# Autodesk Inventor assembly: StorageAssembly.ver4-1111-2020
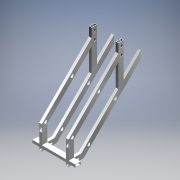
[picture p0: Inventor's stored thumbnail of the model, 180x180]
Saved by Autodesk Inventor 2018 (Build 220112000, 112)
## iProperties
Created: 2020-01-21
Part Number: StorageAssembly.ver4-1111-2020
Document SubType Name: Assembly
Designer: Power Hawks CADD
Author: Power Hawks CADD
## Documents named in this file (7)
- E:\GrabCAD\Power Hawks CAD\2020 Infinite Recharge\Storage\Assemblies\StorageAssembly.ver4-1111-2020.iam
- E:\GrabCAD\Power Hawks CAD\2020 Infinite Recharge\Shooting\Parts\SmallAnglesSupport.ver1-1111-2020.ipt
- E:\GrabCAD\Power Hawks CAD\2020 Infinite Recharge\Shooting\Parts\SmallAnglesSupport.ver1-1111-2020_MIR.ipt
- E:\GrabCAD\Power Hawks CAD\2020 Infinite Recharge\Storage\Assemblies\StorageAssembly.ver3-1111-2020.iam
- E:\GrabCAD\Power Hawks CAD\2020 Infinite Recharge\Storage\Parts\IntakeBrace.ver1-1111-2020.ipt
- E:\GrabCAD\Power Hawks CAD\2020 Infinite Recharge\Storage\Parts\StorageSupport.ver1-1111-2020.ipt
- E:\GrabCAD\Power Hawks CAD\2020 Infinite Recharge\Storage\Parts\AngleBrace.ver2-1111-2020.ipt
## Components (8 placed, 6 different names)
1. SmallAnglesSupport.ver1-1111-2020:1 — Mate:10, Mate:16, Mate:18, Flush:18, Flush:19, Flush:23, Flush:29
2. SmallAnglesSupport.ver1-1111-2020_MIR:1 — Mate:12, Flush:13, Flush:14, Mate:16, Mate:21, Flush:21, Flush:22, Flush:24
3. StorageAssembly.ver3-1111-2020:1 [sub-assembly] — Flush:12, Flush:13, Mate:17, Mate:23, Mate:25, Mate:26
4. IntakeBrace.ver1-1111-2020:1 — Mate:10, Flush:12, Mate:12, Flush:14, Mate:17, Angle:1, Flush:23, Flush:24, Flush:29
5. StorageSupport.ver1-1111-2020:1 — Flush:28, Mate:26, Mate:28
6. StorageSupport.ver1-1111-2020:2 — Flush:27, Mate:25, Mate:27
7. AngleBrace.ver2-1111-2020:1 — Mate:18, Flush:18, Flush:19, Flush:27, Mate:27
8. AngleBrace.ver2-1111-2020:2 — Mate:21, Flush:21, Flush:22, Flush:28, Mate:28
## Relationships (24: Flush 12, Mate 11, Angle 1)
- Mate:10: SmallAnglesSupport.ver1-1111-2020:1 ↔ IntakeBrace.ver1-1111-2020:1
- Flush:12: StorageAssembly.ver3-1111-2020:1 ↔ IntakeBrace.ver1-1111-2020:1
- Mate:12: SmallAnglesSupport.ver1-1111-2020_MIR:1 ↔ IntakeBrace.ver1-1111-2020:1
- Flush:13: SmallAnglesSupport.ver1-1111-2020_MIR:1 ↔ StorageAssembly.ver3-1111-2020:1
- Flush:14: SmallAnglesSupport.ver1-1111-2020_MIR:1 ↔ IntakeBrace.ver1-1111-2020:1
- Mate:16 (228.6 mm): SmallAnglesSupport.ver1-1111-2020:1 ↔ SmallAnglesSupport.ver1-1111-2020_MIR:1
- Mate:17: StorageAssembly.ver3-1111-2020:1 ↔ IntakeBrace.ver1-1111-2020:1
- Mate:18: SmallAnglesSupport.ver1-1111-2020:1 ↔ AngleBrace.ver2-1111-2020:1
- Flush:18: SmallAnglesSupport.ver1-1111-2020:1 ↔ AngleBrace.ver2-1111-2020:1
- Flush:19: SmallAnglesSupport.ver1-1111-2020:1 ↔ AngleBrace.ver2-1111-2020:1
- Mate:21: SmallAnglesSupport.ver1-1111-2020_MIR:1 ↔ AngleBrace.ver2-1111-2020:2
- Flush:21: SmallAnglesSupport.ver1-1111-2020_MIR:1 ↔ AngleBrace.ver2-1111-2020:2
- Flush:22: SmallAnglesSupport.ver1-1111-2020_MIR:1 ↔ AngleBrace.ver2-1111-2020:2
- Angle:1 (0 deg): IntakeBrace.ver1-1111-2020:1
- Flush:23: SmallAnglesSupport.ver1-1111-2020:1 ↔ IntakeBrace.ver1-1111-2020:1
- Flush:24: SmallAnglesSupport.ver1-1111-2020_MIR:1 ↔ IntakeBrace.ver1-1111-2020:1
- Mate:23: StorageAssembly.ver3-1111-2020:1
- Flush:27: StorageSupport.ver1-1111-2020:2 ↔ AngleBrace.ver2-1111-2020:1
- Mate:25: StorageAssembly.ver3-1111-2020:1 ↔ StorageSupport.ver1-1111-2020:2
- Flush:28: StorageSupport.ver1-1111-2020:1 ↔ AngleBrace.ver2-1111-2020:2
- Mate:26: StorageAssembly.ver3-1111-2020:1 ↔ StorageSupport.ver1-1111-2020:1
- Mate:27: StorageSupport.ver1-1111-2020:2 ↔ AngleBrace.ver2-1111-2020:1
- Mate:28: StorageSupport.ver1-1111-2020:1 ↔ AngleBrace.ver2-1111-2020:2
- Flush:29 (63.5 mm): SmallAnglesSupport.ver1-1111-2020:1 ↔ IntakeBrace.ver1-1111-2020:1
